# Autodesk Inventor assembly: Form
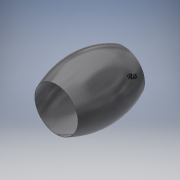
[picture p0: Inventor's stored thumbnail of the model, 180x180]
Saved by Autodesk Inventor 2018.3 (Build 223284000, 284)
## iProperties
Created: 2018-07-24
Part Number: Form
Material: Generisch
Document SubType Name: Assembly
Designer: JochenAlt
Author: JochenAlt
## Documents named in this file (6)
- D:\Projects\FlowerPot\CAD\Form.iam
- D:\Projects\FlowerPot\CAD\Form.ipt
- D:\Projects\FlowerPot\CAD\Spindle\Spindle.ipt
- D:\Projects\FlowerPot\CAD\Spindle\W 61700 X-2RS1.iam
- D:\Projects\FlowerPot\CAD\Spindle\Parallax-Servo_360_Feedback.ipt
- D:\Projects\FlowerPot\CAD\Spindle\BeltPulleyT5_12Z.ipt
## Components (12 placed, 4 different names)
1. Form:1 — Passend:13, Passend:14, Passend:15, Passend:16, Passend:17, Passend:18, Passend:21
2. Spindle:1 — Passend:1, Passend:2, Passend:7, Passend:12, Passend:13
3. Spindle:2 — Passend:3, Passend:4, Passend:8, Passend:11, Passend:14, Fluchtend:2
4. Spindle:3 — Passend:5, Passend:6, Passend:9, Passend:10, Passend:15
5. W 61700 X-2RS1:1 [sub-assembly] — Passend:5, Passend:10, Passend:17
6. W 61700 X-2RS1:2 [sub-assembly] — Passend:6, Passend:9
7. W 61700 X-2RS1:3 [sub-assembly] — Passend:4, Passend:8
8. W 61700 X-2RS1:4 [sub-assembly] — Passend:3, Passend:11, Passend:16
9. W 61700 X-2RS1:5 [sub-assembly] — Passend:2, Passend:7
10. W 61700 X-2RS1:6 [sub-assembly] — Passend:1, Passend:12, Passend:18
11. Parallax-Servo_Feedback:1 — Passend:20
12. Spindle:4 — Passend:20, Fluchtend:2, Passend:21
## Relationships (21: Mate 20, Flush 1)
- Passend:1 [Mate]: Spindle:1 ↔ W 61700 X-2RS1:6
- Passend:2 [Mate]: Spindle:1 ↔ W 61700 X-2RS1:5
- Passend:3 [Mate]: Spindle:2 ↔ W 61700 X-2RS1:4
- Passend:4 [Mate]: Spindle:2 ↔ W 61700 X-2RS1:3
- Passend:5 [Mate]: Spindle:3 ↔ W 61700 X-2RS1:1
- Passend:6 [Mate]: Spindle:3 ↔ W 61700 X-2RS1:2
- Passend:7 [Mate]: Spindle:1 ↔ W 61700 X-2RS1:5
- Passend:8 [Mate]: Spindle:2 ↔ W 61700 X-2RS1:3
- Passend:9 [Mate]: Spindle:3 ↔ W 61700 X-2RS1:2
- Passend:10 [Mate]: Spindle:3 ↔ W 61700 X-2RS1:1
- Passend:11 [Mate]: Spindle:2 ↔ W 61700 X-2RS1:4
- Passend:12 [Mate]: Spindle:1 ↔ W 61700 X-2RS1:6
- Passend:13 [Mate]: Form:1 ↔ Spindle:1
- Passend:14 [Mate]: Form:1 ↔ Spindle:2
- Passend:15 [Mate]: Form:1 ↔ Spindle:3
- Passend:16 [Mate]: Form:1 ↔ W 61700 X-2RS1:4
- Passend:17 [Mate]: Form:1 ↔ W 61700 X-2RS1:1
- Passend:18 [Mate]: Form:1 ↔ W 61700 X-2RS1:6
- Passend:20 [Mate]: Parallax-Servo_Feedback:1 ↔ Spindle:4
- Fluchtend:2 [Flush]: Spindle:2 ↔ Spindle:4
- Passend:21 [Mate]: Form:1 ↔ Spindle:4
